# Autodesk Inventor assembly: Versaplanetery 550 Hex Output
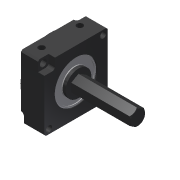
[picture p0: Inventor's stored thumbnail of the model, 180x180]
Saved by Autodesk Inventor 2013 (Build 170138000, 138)
## iProperties
Created: 2013-12-15
Part Number: Versaplanetery 550 Hex Output
Document SubType Name: Assembly
Designer: Nemo
Author: Nemo
## Documents named in this file (5)
- \\lmss\students\Robotics\CAD Files\COTS Parts\VersaPlanetary\Versaplanetery 375 Hex Output.iam
- \\lmss\students\Robotics\CAD Files\COTS Parts\VersaPlanetary\Components\VersaPlanetary Case Shaft Side.ipt
- \\lmss\students\Robotics\CAD Files\COTS Parts\Bearings - VexPro\Radial Bearing - 15mm x 28mm x 7mm.ipt
- \\lmss\students\Robotics\CAD Files\COTS Parts\VersaPlanetary\Components\VersaPlanetary clip ring for shaft.ipt
- \\lmss\students\Robotics\CAD Files\COTS Parts\VersaPlanetary\Components\VersaPlanetary Shaft - 375 Hex.ipt
## Components (5 placed, 4 different names)
1. VersaPlanetary Case Shaft Side:1 — Insert:1, Insert:2, Mate:1, Mate:2, Flush:1
2. Radial Bearing - 15mm x 28mm x 7mm:1 — Insert:2, Insert:3
3. Radial Bearing - 15mm x 28mm x 7mm:2 — Insert:1
4. VersaPlanetary clip ring for shaft:1 — Insert:4
5. VersaPlanetary Shaft - 375 Hex:1 — Insert:3, Insert:4
## Relationships (7: Insert 4, Mate 2, Flush 1)
- Insert:1: VersaPlanetary Case Shaft Side:1 ↔ Radial Bearing - 15mm x 28mm x 7mm:2
- Insert:2: VersaPlanetary Case Shaft Side:1 ↔ Radial Bearing - 15mm x 28mm x 7mm:1
- Insert:3: Radial Bearing - 15mm x 28mm x 7mm:1 ↔ VersaPlanetary Shaft - 375 Hex:1
- Insert:4: VersaPlanetary clip ring for shaft:1 ↔ VersaPlanetary Shaft - 375 Hex:1
- Mate:1: VersaPlanetary Case Shaft Side:1
- Mate:2: VersaPlanetary Case Shaft Side:1
- Flush:1: VersaPlanetary Case Shaft Side:1
